# Autodesk Inventor assembly: C clamp
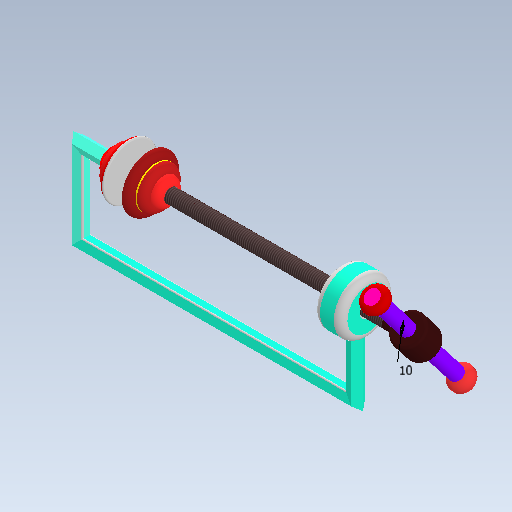
[picture p0: Inventor's stored thumbnail of the model, 512x512]
Saved by Autodesk Inventor 2021 (Build 250183000, 183)
## iProperties
Created: 2021-07-29
Part Number: C clamp
Document SubType Name: Assembly
Designer: Shammy Haider
Author: Shammy Haider
## Documents named in this file (6)
- D:\Designing\Autodesk inventor\C Clamp\C clamp.iam
- D:\Designing\Autodesk inventor\C Clamp\Base.ipt
- D:\Designing\Autodesk inventor\C Clamp\handle.ipt
- D:\Designing\Autodesk inventor\C Clamp\head.ipt
- D:\Designing\Autodesk inventor\C Clamp\knob.ipt
- D:\Designing\Autodesk inventor\C Clamp\rod.ipt
## Components (5 placed, 5 different names)
1. Base:1 — Mate:1
2. handle:1 — Tangent:1, Insert:1, Insert:2, Insert:3
3. head:1 — Mate:2, Mate:3
4. knob:1 — Insert:2, Insert:3
5. rod:1 — Tangent:1, Insert:1, Mate:1, Mate:2, Mate:3
## Relationships (7: Insert 3, Mate 3, Tangent 1)
- Tangent:1: handle:1 ↔ rod:1
- Insert:1 (-38.1 mm): handle:1 ↔ rod:1
- Insert:2: handle:1 ↔ knob:1
- Insert:3: handle:1 ↔ knob:1
- Mate:1: Base:1 ↔ rod:1
- Mate:2: head:1 ↔ rod:1
- Mate:3: head:1 ↔ rod:1
